# Autodesk Inventor assembly: Assembly9 (Crank Case Sub Assembly)
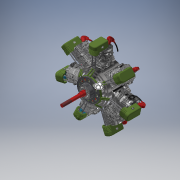
[picture p0: Inventor's stored thumbnail of the model, 180x180]
Saved by Autodesk Inventor 2018 (Build 220112000, 112)
## iProperties
Created: 2023-05-02
Part Number: Assembly9 (Crank Case Sub Assembly)
Document SubType Name: Assembly
Designer: Habib Mohamed
Author: Habib Mohamed
## Documents named in this file (10)
- D:\Inventor\My projects\Rotary Engine\Assembly\Assembly9 (Crank Case Sub Assembly).iam
- D:\Inventor\My projects\Rotary Engine\Main Block (Crank Case).ipt
- D:\Inventor\My projects\Rotary Engine\Assembly\Assembly8 (Cylinder Complete Sub Assembly).iam
- D:\Inventor\My projects\Rotary Engine\Assembly\Assembly6(Piston Sub Assembly Major).iam
- C:\Users\Habib Mohamed\Documents\Inventor\Content Center Files\R2018\en-US\ISO 4762(1)\DIN EN ISO 4762 - M4 x 12.ipt
- D:\Inventor\My projects\Rotary Engine\Assembly\Assembly11 (Cam Sub Assembly).iam
- D:\Inventor\My projects\Rotary Engine\Component 3 (Planet Gear Axis).ipt
- D:\Inventor\My projects\Rotary Engine\Component 20 (Planet Wheel).ipt
- C:\Users\Habib Mohamed\Documents\Inventor\Content Center Files\R2018\en-US\DIN 618 - T1  HK\DIN 618 - HK0609 - 6 x 10 x 9.ipt
- C:\Users\Habib Mohamed\Documents\Inventor\Content Center Files\R2018\en-US\DIN 6799\DIN 6799 - 6 7.ipt
## Components (50 placed, 9 different names)
1. Main Block (Crank Case):1 — Mate:1, Mate:2, Mate:3, Mate:4, Mate:6, Mate:7, Mate:8, Mate:9, Mate:10, Mate:11, Mate:12, Mate:13, Mate:14, Mate:16, Mate:18, Mate:20, Mate:22, Mate:23, Mate:24, Mate:25, Mate:26, Mate:27, Mate:28, Mate:32, Mate:33, Mate:34, Mate:48
2. Assembly6(Piston Sub Assembly Major):1 [sub-assembly] — Mate:1, Mate:5, Mate:6, Mate:7, Mate:8, Mate:9, Mate:10, Mate:11, Mate:12, Mate:47
3. Assembly11 (Cam Sub Assembly):1 [sub-assembly] — Mate:47, Mate:48, Tangent:1, Tangent:2
4. Component 3 (Planet Gear Axis):1 — Mate:23, Mate:26, Mate:29, Mate:35, Mate:36, Mate:41
5. Component 20 (Planet Wheel):1 — Mate:30, Mate:33
6. Component 3 (Planet Gear Axis):2 — Mate:24, Mate:28, Mate:30, Mate:39, Mate:40, Mate:45
7. Component 20 (Planet Wheel):2 — Mate:29, Mate:34
8. Component 3 (Planet Gear Axis):3 — Mate:25, Mate:27, Mate:31, Mate:37, Mate:38, Mate:43
9. Component 20 (Planet Wheel):3 — Mate:31, Mate:32
10. DIN 618 - T1 HK HK0609 - 6 x 10 x 9:1 — Mate:35, Mate:36, Mate:42
11. DIN 618 - T1 HK HK0609 - 6 x 10 x 9:2 — Mate:37, Mate:38, Mate:44
12. DIN 618 - T1 HK HK0609 - 6 x 10 x 9:3 — Mate:39, Mate:40, Mate:46
13. DIN 6799 6:1 — Mate:41, Mate:42
14. DIN 6799 6:2 — Mate:43, Mate:44
15. DIN 6799 6:3 — Mate:45, Mate:46
16. Assembly8 (Cylinder Complete Sub Assembly):1 [sub-assembly] — Mate:2, Mate:3, Mate:4, Mate:5, Mate:13, Mate:15, Mate:17, Mate:19, Mate:21, Tangent:1, Tangent:2
17. DIN EN ISO 4762 M4 x 12:1 — Mate:14, Mate:15
18. DIN EN ISO 4762 M4 x 12:2 — Mate:16, Mate:17
19. DIN EN ISO 4762 M4 x 12:3 — Mate:18, Mate:19
20. DIN EN ISO 4762 M4 x 12:4 — Mate:20, Mate:21
21. Assembly8 (Cylinder Complete Sub Assembly):2 [sub-assembly]
22. DIN EN ISO 4762 M4 x 12:5
23. DIN EN ISO 4762 M4 x 12:6
24. DIN EN ISO 4762 M4 x 12:7
25. DIN EN ISO 4762 M4 x 12:8
26. Assembly8 (Cylinder Complete Sub Assembly):3 [sub-assembly]
27. DIN EN ISO 4762 M4 x 12:9
28. DIN EN ISO 4762 M4 x 12:10
29. DIN EN ISO 4762 M4 x 12:11
30. DIN EN ISO 4762 M4 x 12:12
31. Assembly8 (Cylinder Complete Sub Assembly):4 [sub-assembly]
32. DIN EN ISO 4762 M4 x 12:13
33. DIN EN ISO 4762 M4 x 12:14
34. DIN EN ISO 4762 M4 x 12:15
35. DIN EN ISO 4762 M4 x 12:16
36. Assembly8 (Cylinder Complete Sub Assembly):5 [sub-assembly]
37. DIN EN ISO 4762 M4 x 12:17
38. DIN EN ISO 4762 M4 x 12:18
39. DIN EN ISO 4762 M4 x 12:19
40. DIN EN ISO 4762 M4 x 12:20
41. Assembly8 (Cylinder Complete Sub Assembly):6 [sub-assembly]
42. DIN EN ISO 4762 M4 x 12:21
43. DIN EN ISO 4762 M4 x 12:22
44. DIN EN ISO 4762 M4 x 12:23
45. DIN EN ISO 4762 M4 x 12:24
46. Assembly8 (Cylinder Complete Sub Assembly):7 [sub-assembly]
47. DIN EN ISO 4762 M4 x 12:25
48. DIN EN ISO 4762 M4 x 12:26
49. DIN EN ISO 4762 M4 x 12:27
50. DIN EN ISO 4762 M4 x 12:28
## Component patterns: (7 elements, first: Assembly8 (Cylinder Complete Sub Assembly):1 + DIN EN ISO 4762 M4 x 12:1 + DIN EN ISO 4762 M4 x 12:2 + DIN EN ISO 4762 M4 x 12:3 + DIN EN ISO 4762 M4 x 12:4)
## Relationships (50: Mate 48, Tangent 2)
- Mate:1: Main Block (Crank Case):1 ↔ Assembly6(Piston Sub Assembly Major):1
- Mate:2: Main Block (Crank Case):1 ↔ Assembly8 (Cylinder Complete Sub Assembly):1
- Mate:3: Main Block (Crank Case):1 ↔ Assembly8 (Cylinder Complete Sub Assembly):1
- Mate:4: Main Block (Crank Case):1 ↔ Assembly8 (Cylinder Complete Sub Assembly):1
- Mate:5: Assembly6(Piston Sub Assembly Major):1 ↔ Assembly8 (Cylinder Complete Sub Assembly):1
- Mate:6: Main Block (Crank Case):1 ↔ Assembly6(Piston Sub Assembly Major):1
- Mate:7: Main Block (Crank Case):1 ↔ Assembly6(Piston Sub Assembly Major):1
- Mate:8: Main Block (Crank Case):1 ↔ Assembly6(Piston Sub Assembly Major):1
- Mate:9: Main Block (Crank Case):1 ↔ Assembly6(Piston Sub Assembly Major):1
- Mate:10: Main Block (Crank Case):1 ↔ Assembly6(Piston Sub Assembly Major):1
- Mate:11: Main Block (Crank Case):1 ↔ Assembly6(Piston Sub Assembly Major):1
- Mate:12: Main Block (Crank Case):1 ↔ Assembly6(Piston Sub Assembly Major):1
- Mate:13: Main Block (Crank Case):1 ↔ Assembly8 (Cylinder Complete Sub Assembly):1
- Mate:14: Main Block (Crank Case):1 ↔ DIN EN ISO 4762 M4 x 12:1
- Mate:15: Assembly8 (Cylinder Complete Sub Assembly):1 ↔ DIN EN ISO 4762 M4 x 12:1
- Mate:16: Main Block (Crank Case):1 ↔ DIN EN ISO 4762 M4 x 12:2
- Mate:17: Assembly8 (Cylinder Complete Sub Assembly):1 ↔ DIN EN ISO 4762 M4 x 12:2
- Mate:18: Main Block (Crank Case):1 ↔ DIN EN ISO 4762 M4 x 12:3
- Mate:19: Assembly8 (Cylinder Complete Sub Assembly):1 ↔ DIN EN ISO 4762 M4 x 12:3
- Mate:20: Main Block (Crank Case):1 ↔ DIN EN ISO 4762 M4 x 12:4
- Mate:21: Assembly8 (Cylinder Complete Sub Assembly):1 ↔ DIN EN ISO 4762 M4 x 12:4
- Mate:22: Main Block (Crank Case):1
- Mate:23: Main Block (Crank Case):1 ↔ Component 3 (Planet Gear Axis):1
- Mate:24: Main Block (Crank Case):1 ↔ Component 3 (Planet Gear Axis):2
- Mate:25: Main Block (Crank Case):1 ↔ Component 3 (Planet Gear Axis):3
- Mate:26: Main Block (Crank Case):1 ↔ Component 3 (Planet Gear Axis):1
- Mate:27: Main Block (Crank Case):1 ↔ Component 3 (Planet Gear Axis):3
- Mate:28: Main Block (Crank Case):1 ↔ Component 3 (Planet Gear Axis):2
- Mate:29: Component 3 (Planet Gear Axis):1 ↔ Component 20 (Planet Wheel):2
- Mate:30: Component 20 (Planet Wheel):1 ↔ Component 3 (Planet Gear Axis):2
- Mate:31: Component 3 (Planet Gear Axis):3 ↔ Component 20 (Planet Wheel):3
- Mate:32: Main Block (Crank Case):1 ↔ Component 20 (Planet Wheel):3
- Mate:33: Main Block (Crank Case):1 ↔ Component 20 (Planet Wheel):1
- Mate:34: Main Block (Crank Case):1 ↔ Component 20 (Planet Wheel):2
- Mate:35: Component 3 (Planet Gear Axis):1 ↔ DIN 618 - T1 HK HK0609 - 6 x 10 x 9:1
- Mate:36: Component 3 (Planet Gear Axis):1 ↔ DIN 618 - T1 HK HK0609 - 6 x 10 x 9:1
- Mate:37: Component 3 (Planet Gear Axis):3 ↔ DIN 618 - T1 HK HK0609 - 6 x 10 x 9:2
- Mate:38: Component 3 (Planet Gear Axis):3 ↔ DIN 618 - T1 HK HK0609 - 6 x 10 x 9:2
- Mate:39: Component 3 (Planet Gear Axis):2 ↔ DIN 618 - T1 HK HK0609 - 6 x 10 x 9:3
- Mate:40: Component 3 (Planet Gear Axis):2 ↔ DIN 618 - T1 HK HK0609 - 6 x 10 x 9:3
- Mate:41: Component 3 (Planet Gear Axis):1 ↔ DIN 6799 6:1
- Mate:42: DIN 618 - T1 HK HK0609 - 6 x 10 x 9:1 ↔ DIN 6799 6:1
- Mate:43: Component 3 (Planet Gear Axis):3 ↔ DIN 6799 6:2
- Mate:44: DIN 618 - T1 HK HK0609 - 6 x 10 x 9:2 ↔ DIN 6799 6:2
- Mate:45: Component 3 (Planet Gear Axis):2 ↔ DIN 6799 6:3
- Mate:46: DIN 618 - T1 HK HK0609 - 6 x 10 x 9:3 ↔ DIN 6799 6:3
- Mate:47: Assembly6(Piston Sub Assembly Major):1 ↔ Assembly11 (Cam Sub Assembly):1
- Mate:48: Main Block (Crank Case):1 ↔ Assembly11 (Cam Sub Assembly):1
- Tangent:1: Assembly11 (Cam Sub Assembly):1 ↔ Assembly8 (Cylinder Complete Sub Assembly):1
- Tangent:2: Assembly11 (Cam Sub Assembly):1 ↔ Assembly8 (Cylinder Complete Sub Assembly):1
